# Autodesk Inventor assembly: z_assembly
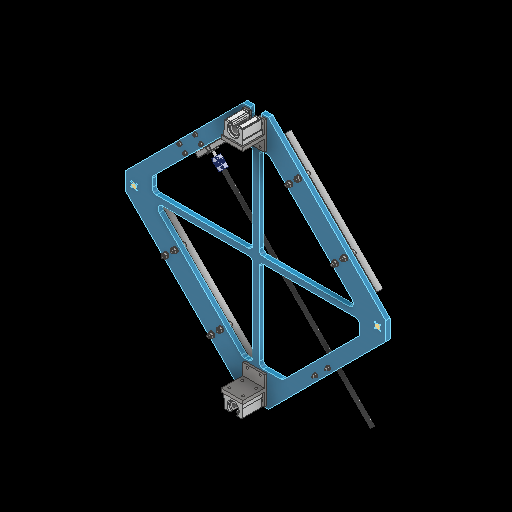
[picture p0: Inventor's stored thumbnail of the model, 512x512]
Saved by Autodesk Inventor 2026.1 (Build 301233000, 233)
## iProperties
Created: 2025-09-21
Part Number: z_assembly
Document SubType Name: Assembly
Designer: drago
Author: drago
## Documents named in this file (19)
- C:\Users\drago\Desktop\_QIST4500_Multidisciplinary_Team_Project\Proteox MX magnet positioner CAD\z_assembly\z_assembly.iam
- C:\Users\drago\Desktop\_QIST4500_Multidisciplinary_Team_Project\Proteox MX magnet positioner CAD\z_assembly\z_plate.ipt
- C:\Users\drago\Desktop\_QIST4500_Multidisciplinary_Team_Project\Proteox MX magnet positioner CAD\z_assembly\x_bearing_bracket.ipt
- C:\Users\drago\Desktop\_QIST4500_Multidisciplinary_Team_Project\Proteox MX magnet positioner CAD\z_assembly\z_bracket.ipt
- C:\Users\drago\Desktop\_QIST4500_Multidisciplinary_Team_Project\Proteox MX magnet positioner CAD\z_assembly\x_rail.ipt
- C:\Users\drago\Desktop\_QIST4500_Multidisciplinary_Team_Project\Proteox MX magnet positioner CAD\z_assembly\x_motor_bracket.ipt
- C:\Users\drago\Desktop\_QIST4500_Multidisciplinary_Team_Project\Proteox MX magnet positioner CAD\other_parts\KP08.iam
- C:\Users\drago\Desktop\_QIST4500_Multidisciplinary_Team_Project\Proteox MX magnet positioner CAD\other_parts\SBR16UU.ipt
- C:\Users\drago\Desktop\_QIST4500_Multidisciplinary_Team_Project\Proteox MX magnet positioner CAD\other_parts\Trapezoidal lead screw Nut tr8x8-4.ipt
- C:\Users\drago\Desktop\_QIST4500_Multidisciplinary_Team_Project\Proteox MX magnet positioner CAD\other_parts\Stepping_Motor_Nema17_34mm.ipt
- C:\Users\drago\Desktop\_QIST4500_Multidisciplinary_Team_Project\Proteox MX magnet positioner CAD\other_parts\5X8_COUPLER.ipt
- C:\Users\drago\Desktop\_QIST4500_Multidisciplinary_Team_Project\Proteox MX magnet positioner CAD\other_parts\Lead Screw 8mm-2.0 x 500mm.ipt
- C:\Users\drago\Documents\Inventor\Content Center Files\R2026\en-US\ISO 7089\ISO 7089 - 4 - 140 HV(1).ipt
- C:\Users\drago\Documents\Inventor\Content Center Files\R2026\en-US\ISO 4762(2)\ISO 4762 - M4 x 30ISO.ipt
- C:\Users\drago\Documents\Inventor\Content Center Files\R2026\en-US\ISO 4032(2)\ISO 4032 - M4 - ISO.ipt
- C:\Users\drago\Documents\Inventor\Content Center Files\R2026\en-US\ISO 4762(2)\ISO 4762 - M4 x 20ISO.ipt
- C:\Users\drago\Documents\Inventor\Content Center Files\R2026\en-US\ISO 7089\ISO 7089 - 6 - 140 HV(1).ipt
- C:\Users\drago\Documents\Inventor\Content Center Files\R2026\en-US\ISO 4032(2)\ISO 4032 - M6 - ISO.ipt
- C:\Users\drago\Documents\Inventor\Content Center Files\R2026\en-US\ISO 4762(2)\ISO 4762 - M6 x 25ISO.ipt
## Components (55 placed, 18 different names)
1. z_plate:1 — Mate:41, Mate:42, Mate:65, Mate:69, Mate:70, Mate:71, Mate:72, Mate:73, Mate:74, Mate:75, Mate:76, Mate:77, Mate:78, Mate:79, Mate:80, Mate:81, Mate:95, Mate:96, Mate:97, Mate:98, Mate:99, Mate:100, Mate:107, Mate:108, Mate:109, Mate:110, Mate:112, Mate:113, Mate:114, Mate:116, Mate:117, Mate:118, Mate:119, Mate:120, Mate:121, Mate:122, Mate:123, Mate:124, Mate:125, Mate:134, Mate:136, Mate:137, Mate:138, Mate:140, Mate:141, Mate:142, Mate:144, Mate:145, Mate:146, Mate:148, Mate:149, Mate:150, Mate:152, Mate:153, Mate:154, Mate:156, Mate:157, Mate:158, Mate:160, Mate:161, Mate:162, Mate:164, Mate:165
2. x_bearing_bracket:1 — Mate:65, Mate:84, Mate:85, Mate:86, Mate:109
3. z_bracket:1 — Mate:75, Mate:77, Mate:78, Mate:87, Mate:89, Mate:90
4. x_rail:1 — Mate:72, Mate:73, Mate:74, Mate:143, Mate:147, Mate:159, Mate:163
5. z_bracket:2 — Mate:76, Mate:79, Mate:80, Mate:88, Mate:91, Mate:92
6. x_rail:2 — Mate:69, Mate:70, Mate:71, Mate:135, Mate:139, Mate:151, Mate:155
7. x_motor_bracket:1 — Mate:81, Mate:101, Mate:102, Mate:103, Mate:107, Mate:108
8. KP08:1 [sub-assembly] — Mate:84, Mate:85, Mate:86, Mate:105, Mate:111, Mate:115
9. SBR16UU:1 — Mate:87, Mate:89, Mate:90
10. SBR16UU:2 — Mate:88, Mate:91, Mate:92
11. Trapezoidal lead screw Nut tr8x8-4:1 — Mate:95, Mate:96, Mate:97
12. Trapezoidal lead screw Nut tr8x8-4:2 — Mate:98, Mate:99, Mate:100
13. Stepping_Motor_Nema17_34mm:1 — Mate:93, Mate:94, Mate:101, Mate:102, Mate:103, Mate:106
14. 5X8_COUPLER:1 — Mate:93, Mate:94, Mate:104
15. Lead Screw 8mm-2.0 x 500mm:1 — Mate:104, Mate:105, Mate:106
16. ISO 7089 4:1 — Mate:110, Mate:111, Insert:1
17. ISO 4762 M4 x 30:1 — Insert:1
18. ISO 7089 4:2 — Mate:112, Mate:113, Insert:2
19. ISO 4032 M4:1 — Insert:2
20. ISO 7089 4:3 — Mate:114, Mate:115, Insert:3
21. ISO 4762 M4 x 30:2 — Insert:3
22. ISO 7089 4:4 — Mate:116, Mate:117, Insert:4
23. ISO 4032 M4:2 — Insert:4
24. ISO 7089 4:5 — Mate:118, Mate:119, Insert:5
25. ISO 4762 M4 x 20:1 — Insert:5
26. ISO 7089 4:6 — Mate:120, Mate:121, Insert:6
27. ISO 4762 M4 x 20:2 — Insert:6
28. ISO 7089 4:7 — Mate:122, Mate:123, Insert:7
29. ISO 4762 M4 x 20:3 — Insert:7
30. ISO 7089 4:8 — Mate:124, Mate:125, Insert:8
31. ISO 4762 M4 x 20:4 — Insert:8
32. ISO 4762 M6 x 25:1 — Mate:134, Mate:135
33. ISO 7089 6:3 — Mate:136, Mate:137, Insert:11
34. ISO 4032 M6:2 — Insert:11
35. ISO 4762 M6 x 25:2 — Mate:138, Mate:139
36. ISO 7089 6:4 — Mate:140, Mate:141, Insert:12
37. ISO 4032 M6:3 — Insert:12
38. ISO 4762 M6 x 25:3 — Mate:142, Mate:143
39. ISO 7089 6:5 — Mate:144, Mate:145, Insert:13
40. ISO 4032 M6:4 — Insert:13
41. ISO 4762 M6 x 25:4 — Mate:146, Mate:147
42. ISO 7089 6:6 — Mate:148, Mate:149, Insert:14
43. ISO 4032 M6:5 — Insert:14
44. ISO 4762 M6 x 25:5 — Mate:150, Mate:151
45. ISO 7089 6:7 — Mate:152, Mate:153, Insert:15
46. ISO 4032 M6:6 — Insert:15
47. ISO 4762 M6 x 25:6 — Mate:154, Mate:155
48. ISO 7089 6:8 — Mate:156, Mate:157, Insert:16
49. ISO 4032 M6:7 — Insert:16
50. ISO 4762 M6 x 25:7 — Mate:158, Mate:159
51. ISO 7089 6:9 — Mate:160, Mate:161, Insert:17
52. ISO 4032 M6:8 — Insert:17
53. ISO 4762 M6 x 25:8 — Mate:162, Mate:163
54. ISO 7089 6:10 — Mate:164, Mate:165, Insert:18
55. ISO 4032 M6:9 — Insert:18
## Relationships (106: Mate 90, Insert 16)
- Mate:41: z_plate:1
- Mate:42: z_plate:1
- Mate:65: z_plate:1 ↔ x_bearing_bracket:1
- Mate:69: z_plate:1 ↔ x_rail:2
- Mate:70: z_plate:1 ↔ x_rail:2
- Mate:71: z_plate:1 ↔ x_rail:2
- Mate:72: z_plate:1 ↔ x_rail:1
- Mate:73: z_plate:1 ↔ x_rail:1
- Mate:74: z_plate:1 ↔ x_rail:1
- Mate:75: z_plate:1 ↔ z_bracket:1
- Mate:76: z_plate:1 ↔ z_bracket:2
- Mate:77: z_plate:1 ↔ z_bracket:1
- Mate:78: z_plate:1 ↔ z_bracket:1
- Mate:79: z_plate:1 ↔ z_bracket:2
- Mate:80: z_plate:1 ↔ z_bracket:2
- Mate:81: z_plate:1 ↔ x_motor_bracket:1
- Mate:84: x_bearing_bracket:1 ↔ KP08:1
- Mate:85: x_bearing_bracket:1 ↔ KP08:1
- Mate:86: x_bearing_bracket:1 ↔ KP08:1
- Mate:87: z_bracket:1 ↔ SBR16UU:1
- Mate:88: z_bracket:2 ↔ SBR16UU:2
- Mate:89: z_bracket:1 ↔ SBR16UU:1
- Mate:90: z_bracket:1 ↔ SBR16UU:1
- Mate:91: z_bracket:2 ↔ SBR16UU:2
- Mate:92: z_bracket:2 ↔ SBR16UU:2
- Mate:93: Stepping_Motor_Nema17_34mm:1 ↔ 5X8_COUPLER:1
- Mate:94 (10 mm): Stepping_Motor_Nema17_34mm:1 ↔ 5X8_COUPLER:1
- Mate:95: z_plate:1 ↔ Trapezoidal lead screw Nut tr8x8-4:1
- Mate:96: z_plate:1 ↔ Trapezoidal lead screw Nut tr8x8-4:1
- Mate:97: z_plate:1 ↔ Trapezoidal lead screw Nut tr8x8-4:1
- Mate:98: z_plate:1 ↔ Trapezoidal lead screw Nut tr8x8-4:2
- Mate:99: z_plate:1 ↔ Trapezoidal lead screw Nut tr8x8-4:2
- Mate:100: z_plate:1 ↔ Trapezoidal lead screw Nut tr8x8-4:2
- Mate:101: x_motor_bracket:1 ↔ Stepping_Motor_Nema17_34mm:1
- Mate:102: x_motor_bracket:1 ↔ Stepping_Motor_Nema17_34mm:1
- Mate:103: x_motor_bracket:1 ↔ Stepping_Motor_Nema17_34mm:1
- Mate:104: 5X8_COUPLER:1 ↔ Lead Screw 8mm-2.0 x 500mm:1
- Mate:105: KP08:1 ↔ Lead Screw 8mm-2.0 x 500mm:1
- Mate:106: Stepping_Motor_Nema17_34mm:1 ↔ Lead Screw 8mm-2.0 x 500mm:1
- Mate:107: z_plate:1 ↔ x_motor_bracket:1
- Mate:108: z_plate:1 ↔ x_motor_bracket:1
- Mate:109: z_plate:1 ↔ x_bearing_bracket:1
- Mate:110: z_plate:1 ↔ ISO 7089 4:1
- Mate:111: KP08:1 ↔ ISO 7089 4:1
- Insert:1: ISO 7089 4:1 ↔ ISO 4762 M4 x 30:1
- Mate:112: z_plate:1 ↔ ISO 7089 4:2
- Mate:113: z_plate:1 ↔ ISO 7089 4:2
- Insert:2: ISO 7089 4:2 ↔ ISO 4032 M4:1
- Mate:114: z_plate:1 ↔ ISO 7089 4:3
- Mate:115: KP08:1 ↔ ISO 7089 4:3
- Insert:3: ISO 7089 4:3 ↔ ISO 4762 M4 x 30:2
- Mate:116: z_plate:1 ↔ ISO 7089 4:4
- Mate:117: z_plate:1 ↔ ISO 7089 4:4
- Insert:4: ISO 7089 4:4 ↔ ISO 4032 M4:2
- Mate:118: z_plate:1 ↔ ISO 7089 4:5
- Mate:119: z_plate:1 ↔ ISO 7089 4:5
- Insert:5: ISO 7089 4:5 ↔ ISO 4762 M4 x 20:1
- Mate:120: z_plate:1 ↔ ISO 7089 4:6
- Mate:121: z_plate:1 ↔ ISO 7089 4:6
- Insert:6: ISO 7089 4:6 ↔ ISO 4762 M4 x 20:2
- Mate:122: z_plate:1 ↔ ISO 7089 4:7
- Mate:123: z_plate:1 ↔ ISO 7089 4:7
- Insert:7: ISO 7089 4:7 ↔ ISO 4762 M4 x 20:3
- Mate:124: z_plate:1 ↔ ISO 7089 4:8
- Mate:125: z_plate:1 ↔ ISO 7089 4:8
- Insert:8: ISO 7089 4:8 ↔ ISO 4762 M4 x 20:4
- Mate:134: z_plate:1 ↔ ISO 4762 M6 x 25:1
- Mate:135: x_rail:2 ↔ ISO 4762 M6 x 25:1
- Mate:136: z_plate:1 ↔ ISO 7089 6:3
- Mate:137: z_plate:1 ↔ ISO 7089 6:3
- Insert:11: ISO 7089 6:3 ↔ ISO 4032 M6:2
- Mate:138: z_plate:1 ↔ ISO 4762 M6 x 25:2
- Mate:139: x_rail:2 ↔ ISO 4762 M6 x 25:2
- Mate:140: z_plate:1 ↔ ISO 7089 6:4
- Mate:141: z_plate:1 ↔ ISO 7089 6:4
- Insert:12: ISO 7089 6:4 ↔ ISO 4032 M6:3
- Mate:142: z_plate:1 ↔ ISO 4762 M6 x 25:3
- Mate:143: x_rail:1 ↔ ISO 4762 M6 x 25:3
- Mate:144: z_plate:1 ↔ ISO 7089 6:5
- Mate:145: z_plate:1 ↔ ISO 7089 6:5
- Insert:13: ISO 7089 6:5 ↔ ISO 4032 M6:4
- Mate:146: z_plate:1 ↔ ISO 4762 M6 x 25:4
- Mate:147: x_rail:1 ↔ ISO 4762 M6 x 25:4
- Mate:148: z_plate:1 ↔ ISO 7089 6:6
- Mate:149: z_plate:1 ↔ ISO 7089 6:6
- Insert:14: ISO 7089 6:6 ↔ ISO 4032 M6:5
- Mate:150: z_plate:1 ↔ ISO 4762 M6 x 25:5
- Mate:151: x_rail:2 ↔ ISO 4762 M6 x 25:5
- Mate:152: z_plate:1 ↔ ISO 7089 6:7
- Mate:153: z_plate:1 ↔ ISO 7089 6:7
- Insert:15: ISO 7089 6:7 ↔ ISO 4032 M6:6
- Mate:154: z_plate:1 ↔ ISO 4762 M6 x 25:6
- Mate:155: x_rail:2 ↔ ISO 4762 M6 x 25:6
- Mate:156: z_plate:1 ↔ ISO 7089 6:8
- Mate:157: z_plate:1 ↔ ISO 7089 6:8
- Insert:16: ISO 7089 6:8 ↔ ISO 4032 M6:7
- Mate:158: z_plate:1 ↔ ISO 4762 M6 x 25:7
- Mate:159: x_rail:1 ↔ ISO 4762 M6 x 25:7
- Mate:160: z_plate:1 ↔ ISO 7089 6:9
- Mate:161: z_plate:1 ↔ ISO 7089 6:9
- Insert:17: ISO 7089 6:9 ↔ ISO 4032 M6:8
- Mate:162: z_plate:1 ↔ ISO 4762 M6 x 25:8
- Mate:163: x_rail:1 ↔ ISO 4762 M6 x 25:8
- Mate:164: z_plate:1 ↔ ISO 7089 6:10
- Mate:165: z_plate:1 ↔ ISO 7089 6:10
- Insert:18: ISO 7089 6:10 ↔ ISO 4032 M6:9
